# Autodesk Inventor assembly: Trunk
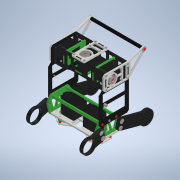
[picture p0: Inventor's stored thumbnail of the model, 180x180]
Saved by Autodesk Inventor 2020.4 (Build 244396000, 396)
## iProperties
Created: 2022-01-05
Part Number: Trunk
Document SubType Name: Assembly
Designer: Masato Kubotera
Mass: 836.462 g
Surface Area: 2738.45 cm^2
Volume: 519.507 cm^3
Density: 1.61011 g/cm^3
Author: Masato Kubotera
## Documents named in this file (24)
- C:\Users\Masato\Desktop\SUSTAINA-OP\UpperBody\Trunk\Trunk.iam
- C:\Users\Masato\Desktop\SUSTAINA-OP\ReadyMade\KONDO\B3M-SC-1170-A.ipt
- C:\Users\Masato\Desktop\SUSTAINA-OP\UpperBody\Trunk\Trunk_chest_frame.ipt
- C:\Users\Masato\Desktop\SUSTAINA-OP\ReadyMade\InsertNut\IRU-304SW.ipt
- C:\Users\Masato\Desktop\SUSTAINA-OP\UpperBody\Trunk\Trunk_neck_frame.ipt
- C:\Users\Masato\Desktop\SUSTAINA-OP\ReadyMade\Screw\M2_6-15.ipt
- C:\Users\Masato\Desktop\SUSTAINA-OP\ReadyMade\Screw\M3-6.ipt
- C:\Users\Masato\Desktop\SUSTAINA-OP\ReadyMade\Screw\M3-8.ipt
- C:\Users\Masato\Desktop\SUSTAINA-OP\UpperBody\Trunk\Trunk_shoulder_frame.ipt
- C:\Users\Masato\Desktop\SUSTAINA-OP\UpperBody\Trunk\Trunk_upper_side_frame.ipt
- C:\Users\Masato\Desktop\SUSTAINA-OP\ReadyMade\Screw\M3-10.ipt
- C:\Users\Masato\Desktop\SUSTAINA-OP\UpperBody\Trunk\Trunk_shoulder_frame_MIR.ipt
- C:\Users\Masato\Desktop\SUSTAINA-OP\ReadyMade\Washer\UUW-0312-10H.ipt
- C:\Users\Masato\Desktop\SUSTAINA-OP\UpperBody\Trunk\Trunk_lower_side_frame.ipt
- C:\Users\Masato\Desktop\SUSTAINA-OP\UpperBody\Trunk\Trunk_waisit_frame.ipt
- C:\Users\Masato\Desktop\SUSTAINA-OP\UpperBody\Trunk\CrossRollerBearing\BearingUnit.iam
- C:\Users\Masato\Desktop\SUSTAINA-OP\ReadyMade\Screw\SPNFL-BRN-M3-6.ipt
- C:\Users\Masato\Desktop\SUSTAINA-OP\ReadyMade\Spacer\ABLSBF7-140-M3-N3.ipt
- C:\Users\Masato\Desktop\SUSTAINA-OP\ReadyMade\Spacer\ABLSBF7-157-M3-N3.ipt
- C:\Users\Masato\Desktop\SUSTAINA-OP\ReadyMade\Spacer\BRU-309S.ipt
- C:\Users\Masato\Desktop\SUSTAINA-OP\UpperBody\Trunk\Trunk_servo_bottom_frame.ipt
- C:\Users\Masato\Desktop\SUSTAINA-OP\ReadyMade\KONDO\B3M-SC-1040-A_with_ClampHorn.iam
- C:\Users\Masato\Desktop\SUSTAINA-OP\UpperBody\Trunk\FrontBumper.ipt
- C:\Users\Masato\Desktop\SUSTAINA-OP\UpperBody\Trunk\RearBumper.ipt
## Components (101 placed, 23 different names)
1. B3M-SC-1170-A:1 — 挿入:87, 挿入:88
2. B3M-SC-1170-A:2 — 挿入:89, 挿入:90
3. Trunk_chest_frame:1 — 挿入:2, 挿入:3, 挿入:4, 挿入:6, 挿入:131
4. Trunk_chest_frame:2 — 挿入:7, 挿入:9, 挿入:10, 挿入:11, 挿入:12, 挿入:8
5. Trunk_neck_frame:1 — 挿入:18, 挿入:20, 挿入:25, 挿入:26, 挿入:27, 挿入:28, 挿入:202, 挿入:203, 挿入:204, 挿入:205
6. Trunk_upper_side_frame:1 — 挿入:29, 挿入:30, 挿入:31, 挿入:32, 挿入:33, 挿入:34, 挿入:35, 挿入:36, 挿入:5, 挿入:119, 挿入:189, 挿入:190, 挿入:193, 挿入:195, 挿入:196
7. Trunk_shoulder_frame:1 — 挿入:33, 挿入:34, 挿入:35, 挿入:36, 挿入:37, 挿入:39, 挿入:38, 挿入:40, 挿入:139, 挿入:200, 挿入:201, 挿入:206, 挿入:207
8. Trunk_upper_side_frame:2 — 挿入:52, 挿入:53, 挿入:54, 挿入:55, 挿入:56, 挿入:57, 挿入:58, 挿入:59, 挿入:120, 挿入:191, 挿入:192, 挿入:194
9. Trunk_shoulder_frame_MIR:1 — 挿入:56, 挿入:57, 挿入:58, 挿入:59, 挿入:65, 挿入:66, 挿入:67, 挿入:68, 挿入:71, 挿入:72, 角度:5, 挿入:141, 挿入:208, 挿入:209
10. UUW-0312-10H:1 — 挿入:75, 挿入:140
11. UUW-0312-10H:2 — 挿入:76, 挿入:142
12. Trunk_lower_side_frame:1 — 挿入:177, 挿入:178, 角度:6, 角度:7, 挿入:179, 挿入:180, 挿入:195, 挿入:196, 挿入:214, 挿入:215, 挿入:216, 挿入:217
13. Trunk_lower_side_frame:2 — 挿入:143, 挿入:144, 挿入:210, 挿入:211, 挿入:212, 挿入:213
14. Trunk_waisit_frame:1 — フラッシュ:2, フラッシュ:3, フラッシュ:4, 挿入:83, 挿入:84, 挿入:85, 挿入:86, 挿入:87, 挿入:88, 挿入:89, 挿入:90, 挿入:91, 挿入:92, 挿入:93, 挿入:94, 挿入:121, 挿入:122, 挿入:123, 挿入:124, 挿入:143, 挿入:144, 挿入:177, 挿入:178
15. BearingUnit:1 [sub-assembly] — 挿入:83, 挿入:84
16. BearingUnit:2 [sub-assembly] — 挿入:85, 挿入:86
17. ABLSBF7-140-M3-N3:1 — 角度:6, 挿入:179
18. ABLSBF7-140-M3-N3:2 — 角度:7, 挿入:180
19. ABLSBF7-157-M3-N3:1 — 角度:5, 挿入:139, 挿入:140, 挿入:141, 挿入:142
20. BRU-309S:1 — 挿入:161, 挿入:214
21. BRU-309S:2 — 挿入:162, 挿入:215
22. BRU-309S:3 — 挿入:163, 挿入:216
23. BRU-309S:4 — 挿入:164, 挿入:217
24. BRU-309S:5 — 挿入:165, 挿入:210
25. BRU-309S:6 — 挿入:166, 挿入:211
26. BRU-309S:7 — 挿入:167, 挿入:212
27. BRU-309S:8 — 挿入:168, 挿入:213
28. UUW-0312-10H:11 — 挿入:161, 挿入:169, 挿入:218
29. UUW-0312-10H:12 — 挿入:162, 挿入:170, 挿入:219
30. UUW-0312-10H:13 — 挿入:163, 挿入:171, 挿入:220
31. UUW-0312-10H:14 — 挿入:164, 挿入:172, 挿入:221
32. UUW-0312-10H:15 — 挿入:165, 挿入:173, 挿入:224
33. UUW-0312-10H:16 — 挿入:166, 挿入:174, 挿入:225
34. UUW-0312-10H:17 — 挿入:167, 挿入:175, 挿入:222
35. UUW-0312-10H:18 — 挿入:168, 挿入:176, 挿入:223
36. Trunk_servo_bottom_frame:1
37. Trunk_servo_bottom_frame:2
38. Trunk_servo_bottom_frame:3
39. M2_6-15:19 — 挿入:202
40. M2_6-15:20 — 挿入:203
41. B3M-SC-1040-A_with_ClampHorn:1 [sub-assembly] — 挿入:204, 挿入:205
42. B3M-SC-1040-A_with_ClampHorn:2 [sub-assembly] — 挿入:206, 挿入:207
43. B3M-SC-1040-A_with_ClampHorn:3 [sub-assembly] — 挿入:208, 挿入:209
44. FrontBumper:1 — 挿入:218, 挿入:219
45. RearBumper:1 — 挿入:220, 挿入:221
46. FrontBumper:2 — 挿入:222, 挿入:223
47. RearBumper:2 — 挿入:224, 挿入:225
48. M2_6-15:17 — 挿入:201
49. M2_6-15:18 — 挿入:200
50. M3-6:9 — 挿入:169
51. M3-6:10 — 挿入:170
52. M3-6:11 — 挿入:171
53. M3-6:12 — 挿入:172
54. M3-6:13 — 挿入:173
55. M3-6:14 — 挿入:174
56. M3-6:15 — 挿入:176
57. M3-6:16 — 挿入:175
58. M3-10:17 — 挿入:189
59. M3-10:18 — 挿入:190
60. M3-10:19 — 挿入:191
61. M3-10:20 — 挿入:192
62. M3-8:7 — 挿入:193
63. M3-8:8 — 挿入:194
64. M3-10:13 — 挿入:121
65. M3-10:14 — 挿入:122
66. M3-10:15 — 挿入:123
67. M3-10:16 — 挿入:124
68. SPNFL-BRN-M3-6:1 — 挿入:119
69. SPNFL-BRN-M3-6:2 — 挿入:120
70. M3-8:2 — 挿入:28
71. M3-8:1 — 挿入:27
72. M3-6:2 — 挿入:26
73. M3-6:1 — 挿入:25
74. M3-8:4 — 挿入:38
75. M3-8:3 — 挿入:37
76. M3-10:4 — 挿入:40
77. M3-10:3 — 挿入:39
78. M2_6-15:12 — 挿入:72
79. M2_6-15:11 — 挿入:71
80. M3-10:6 — 挿入:68
81. M3-10:5 — 挿入:67
82. M3-8:6 — 挿入:66
83. M3-8:5 — 挿入:65
84. M3-6:4 — 挿入:76
85. M3-6:3 — 挿入:75
86. M2_6-15:16 — 挿入:94
87. M2_6-15:15 — 挿入:93
88. M2_6-15:14 — 挿入:92
89. M2_6-15:13 — 挿入:91
90. IRU-304SW:12 — 挿入:12, 挿入:53
91. IRU-304SW:11 — 挿入:11, 挿入:52
92. IRU-304SW:10 — 挿入:10, 挿入:30
93. IRU-304SW:9 — 挿入:9, 挿入:29
94. IRU-304SW:8 — 挿入:8
95. IRU-304SW:7 — 挿入:7, 挿入:18
96. IRU-304SW:6 — 挿入:6, 挿入:32
97. IRU-304SW:5 — 挿入:5, 挿入:31
98. IRU-304SW:4 — 挿入:4, 挿入:55
99. IRU-304SW:3 — 挿入:3, 挿入:54
100. IRU-304SW:2 — 挿入:2, 挿入:20
101. IRU-304SW:1 — 挿入:131
## Relationships (130: Insert 124, Flush 3, Angle 3)
- 挿入:2 [Insert]: Trunk_chest_frame:1 ↔ IRU-304SW:2
- 挿入:3 [Insert]: Trunk_chest_frame:1 ↔ IRU-304SW:3
- 挿入:4 [Insert]: Trunk_chest_frame:1 ↔ IRU-304SW:4
- 挿入:5 [Insert]: Trunk_upper_side_frame:1 ↔ IRU-304SW:5
- 挿入:6 [Insert]: Trunk_chest_frame:1 ↔ IRU-304SW:6
- 挿入:7 [Insert]: Trunk_chest_frame:2 ↔ IRU-304SW:7
- 挿入:8 [Insert]: Trunk_chest_frame:2 ↔ IRU-304SW:8
- 挿入:9 [Insert]: Trunk_chest_frame:2 ↔ IRU-304SW:9
- 挿入:10 [Insert]: Trunk_chest_frame:2 ↔ IRU-304SW:10
- 挿入:11 [Insert]: Trunk_chest_frame:2 ↔ IRU-304SW:11
- 挿入:12 [Insert]: Trunk_chest_frame:2 ↔ IRU-304SW:12
- 挿入:18 [Insert]: Trunk_neck_frame:1 ↔ IRU-304SW:7
- 挿入:20 [Insert]: Trunk_neck_frame:1 ↔ IRU-304SW:2
- 挿入:25 [Insert]: Trunk_neck_frame:1 ↔ M3-6:1
- 挿入:26 [Insert]: Trunk_neck_frame:1 ↔ M3-6:2
- 挿入:27 [Insert]: Trunk_neck_frame:1 ↔ M3-8:1
- 挿入:28 [Insert]: Trunk_neck_frame:1 ↔ M3-8:2
- 挿入:29 [Insert]: Trunk_upper_side_frame:1 ↔ IRU-304SW:9
- 挿入:30 [Insert]: Trunk_upper_side_frame:1 ↔ IRU-304SW:10
- 挿入:31 [Insert]: Trunk_upper_side_frame:1 ↔ IRU-304SW:5
- 挿入:32 [Insert]: Trunk_upper_side_frame:1 ↔ IRU-304SW:6
- 挿入:33 [Insert]: Trunk_upper_side_frame:1 ↔ Trunk_shoulder_frame:1
- 挿入:34 [Insert]: Trunk_upper_side_frame:1 ↔ Trunk_shoulder_frame:1
- 挿入:35 [Insert]: Trunk_upper_side_frame:1 ↔ Trunk_shoulder_frame:1
- 挿入:36 [Insert]: Trunk_upper_side_frame:1 ↔ Trunk_shoulder_frame:1
- 挿入:37 [Insert]: Trunk_shoulder_frame:1 ↔ M3-8:3
- 挿入:39 [Insert]: Trunk_shoulder_frame:1 ↔ M3-10:3
- 挿入:38 [Insert]: Trunk_shoulder_frame:1 ↔ M3-8:4
- 挿入:40 [Insert]: Trunk_shoulder_frame:1 ↔ M3-10:4
- 挿入:52 [Insert]: Trunk_upper_side_frame:2 ↔ IRU-304SW:11
- 挿入:53 [Insert]: Trunk_upper_side_frame:2 ↔ IRU-304SW:12
- 挿入:54 [Insert]: Trunk_upper_side_frame:2 ↔ IRU-304SW:3
- 挿入:55 [Insert]: Trunk_upper_side_frame:2 ↔ IRU-304SW:4
- 挿入:56 [Insert]: Trunk_upper_side_frame:2 ↔ Trunk_shoulder_frame_MIR:1
- 挿入:57 [Insert]: Trunk_upper_side_frame:2 ↔ Trunk_shoulder_frame_MIR:1
- 挿入:58 [Insert]: Trunk_upper_side_frame:2 ↔ Trunk_shoulder_frame_MIR:1
- 挿入:59 [Insert]: Trunk_upper_side_frame:2 ↔ Trunk_shoulder_frame_MIR:1
- 挿入:65 [Insert]: Trunk_shoulder_frame_MIR:1 ↔ M3-8:5
- 挿入:66 [Insert]: Trunk_shoulder_frame_MIR:1 ↔ M3-8:6
- 挿入:67 [Insert]: Trunk_shoulder_frame_MIR:1 ↔ M3-10:5
- 挿入:68 [Insert]: Trunk_shoulder_frame_MIR:1 ↔ M3-10:6
- 挿入:71 [Insert]: Trunk_shoulder_frame_MIR:1 ↔ M2_6-15:11
- 挿入:72 [Insert]: Trunk_shoulder_frame_MIR:1 ↔ M2_6-15:12
- 挿入:75 [Insert]: UUW-0312-10H:1 ↔ M3-6:3
- 挿入:76 [Insert]: UUW-0312-10H:2 ↔ M3-6:4
- フラッシュ:2 [Flush]: Trunk_waisit_frame:1
- フラッシュ:3 [Flush]: Trunk_waisit_frame:1
- フラッシュ:4 [Flush]: Trunk_waisit_frame:1
- 挿入:83 [Insert]: Trunk_waisit_frame:1 ↔ BearingUnit:1
- 挿入:84 [Insert]: Trunk_waisit_frame:1 ↔ BearingUnit:1
- 挿入:85 [Insert]: Trunk_waisit_frame:1 ↔ BearingUnit:2
- 挿入:86 [Insert]: Trunk_waisit_frame:1 ↔ BearingUnit:2
- 挿入:87 [Insert]: B3M-SC-1170-A:1 ↔ Trunk_waisit_frame:1
- 挿入:88 [Insert]: B3M-SC-1170-A:1 ↔ Trunk_waisit_frame:1
- 挿入:89 [Insert]: B3M-SC-1170-A:2 ↔ Trunk_waisit_frame:1
- 挿入:90 [Insert]: B3M-SC-1170-A:2 ↔ Trunk_waisit_frame:1
- 挿入:91 [Insert]: Trunk_waisit_frame:1 ↔ M2_6-15:13
- 挿入:92 [Insert]: Trunk_waisit_frame:1 ↔ M2_6-15:14
- 挿入:93 [Insert]: Trunk_waisit_frame:1 ↔ M2_6-15:15
- 挿入:94 [Insert]: Trunk_waisit_frame:1 ↔ M2_6-15:16
- 挿入:119 [Insert]: Trunk_upper_side_frame:1 ↔ SPNFL-BRN-M3-6:1
- 挿入:120 [Insert]: Trunk_upper_side_frame:2 ↔ SPNFL-BRN-M3-6:2
- 挿入:121 [Insert]: Trunk_waisit_frame:1 ↔ M3-10:13
- 挿入:122 [Insert]: Trunk_waisit_frame:1 ↔ M3-10:14
- 挿入:123 [Insert]: Trunk_waisit_frame:1 ↔ M3-10:15
- 挿入:124 [Insert]: Trunk_waisit_frame:1 ↔ M3-10:16
- 挿入:131 [Insert]: Trunk_chest_frame:1 ↔ IRU-304SW:1
- 角度:5 [Angle] (0 deg): Trunk_shoulder_frame_MIR:1 ↔ ABLSBF7-157-M3-N3:1
- 挿入:139 [Insert]: Trunk_shoulder_frame:1 ↔ ABLSBF7-157-M3-N3:1
- 挿入:140 [Insert]: UUW-0312-10H:1 ↔ ABLSBF7-157-M3-N3:1
- 挿入:141 [Insert]: Trunk_shoulder_frame_MIR:1 ↔ ABLSBF7-157-M3-N3:1
- 挿入:142 [Insert]: UUW-0312-10H:2 ↔ ABLSBF7-157-M3-N3:1
- 挿入:143 [Insert]: Trunk_lower_side_frame:2 ↔ Trunk_waisit_frame:1
- 挿入:144 [Insert]: Trunk_lower_side_frame:2 ↔ Trunk_waisit_frame:1
- 挿入:161 [Insert]: BRU-309S:1 ↔ UUW-0312-10H:11
- 挿入:162 [Insert]: BRU-309S:2 ↔ UUW-0312-10H:12
- 挿入:163 [Insert]: BRU-309S:3 ↔ UUW-0312-10H:13
- 挿入:164 [Insert]: BRU-309S:4 ↔ UUW-0312-10H:14
- 挿入:165 [Insert]: BRU-309S:5 ↔ UUW-0312-10H:15
- 挿入:166 [Insert]: BRU-309S:6 ↔ UUW-0312-10H:16
- 挿入:167 [Insert]: BRU-309S:7 ↔ UUW-0312-10H:17
- 挿入:168 [Insert]: BRU-309S:8 ↔ UUW-0312-10H:18
- 挿入:169 [Insert]: UUW-0312-10H:11 ↔ M3-6:9
- 挿入:170 [Insert]: UUW-0312-10H:12 ↔ M3-6:10
- 挿入:171 [Insert]: UUW-0312-10H:13 ↔ M3-6:11
- 挿入:172 [Insert]: UUW-0312-10H:14 ↔ M3-6:12
- 挿入:173 [Insert]: UUW-0312-10H:15 ↔ M3-6:13
- 挿入:174 [Insert]: UUW-0312-10H:16 ↔ M3-6:14
- 挿入:175 [Insert]: UUW-0312-10H:17 ↔ M3-6:16
- 挿入:176 [Insert]: UUW-0312-10H:18 ↔ M3-6:15
- 挿入:177 [Insert]: Trunk_lower_side_frame:1 ↔ Trunk_waisit_frame:1
- 挿入:178 [Insert]: Trunk_lower_side_frame:1 ↔ Trunk_waisit_frame:1
- 角度:6 [Angle] (0 deg): Trunk_lower_side_frame:1 ↔ ABLSBF7-140-M3-N3:1
- 角度:7 [Angle] (0 deg): Trunk_lower_side_frame:1 ↔ ABLSBF7-140-M3-N3:2
- 挿入:179 [Insert]: Trunk_lower_side_frame:1 ↔ ABLSBF7-140-M3-N3:1
- 挿入:180 [Insert]: Trunk_lower_side_frame:1 ↔ ABLSBF7-140-M3-N3:2
- 挿入:189 [Insert]: Trunk_upper_side_frame:1 ↔ M3-10:17
- 挿入:190 [Insert]: Trunk_upper_side_frame:1 ↔ M3-10:18
- 挿入:191 [Insert]: Trunk_upper_side_frame:2 ↔ M3-10:19
- 挿入:192 [Insert]: Trunk_upper_side_frame:2 ↔ M3-10:20
- 挿入:193 [Insert]: Trunk_upper_side_frame:1 ↔ M3-8:7
- 挿入:194 [Insert]: Trunk_upper_side_frame:2 ↔ M3-8:8
- 挿入:195 [Insert]: Trunk_upper_side_frame:1 ↔ Trunk_lower_side_frame:1
- 挿入:196 [Insert]: Trunk_upper_side_frame:1 ↔ Trunk_lower_side_frame:1
- 挿入:200 [Insert]: Trunk_shoulder_frame:1 ↔ M2_6-15:18
- 挿入:201 [Insert]: Trunk_shoulder_frame:1 ↔ M2_6-15:17
- 挿入:202 [Insert]: Trunk_neck_frame:1 ↔ M2_6-15:19
- 挿入:203 [Insert]: Trunk_neck_frame:1 ↔ M2_6-15:20
- 挿入:204 [Insert]: Trunk_neck_frame:1 ↔ B3M-SC-1040-A_with_ClampHorn:1
- 挿入:205 [Insert]: Trunk_neck_frame:1 ↔ B3M-SC-1040-A_with_ClampHorn:1
- 挿入:206 [Insert]: Trunk_shoulder_frame:1 ↔ B3M-SC-1040-A_with_ClampHorn:2
- 挿入:207 [Insert]: Trunk_shoulder_frame:1 ↔ B3M-SC-1040-A_with_ClampHorn:2
- 挿入:208 [Insert]: Trunk_shoulder_frame_MIR:1 ↔ B3M-SC-1040-A_with_ClampHorn:3
- 挿入:209 [Insert]: Trunk_shoulder_frame_MIR:1 ↔ B3M-SC-1040-A_with_ClampHorn:3
- 挿入:210 [Insert]: Trunk_lower_side_frame:2 ↔ BRU-309S:5
- 挿入:211 [Insert]: Trunk_lower_side_frame:2 ↔ BRU-309S:6
- 挿入:212 [Insert]: Trunk_lower_side_frame:2 ↔ BRU-309S:7
- 挿入:213 [Insert]: Trunk_lower_side_frame:2 ↔ BRU-309S:8
- 挿入:214 [Insert]: Trunk_lower_side_frame:1 ↔ BRU-309S:1
- 挿入:215 [Insert]: Trunk_lower_side_frame:1 ↔ BRU-309S:2
- 挿入:216 [Insert]: Trunk_lower_side_frame:1 ↔ BRU-309S:3
- 挿入:217 [Insert]: Trunk_lower_side_frame:1 ↔ BRU-309S:4
- 挿入:218 [Insert]: UUW-0312-10H:11 ↔ FrontBumper:1
- 挿入:219 [Insert]: UUW-0312-10H:12 ↔ FrontBumper:1
- 挿入:220 [Insert]: UUW-0312-10H:13 ↔ RearBumper:1
- 挿入:221 [Insert]: UUW-0312-10H:14 ↔ RearBumper:1
- 挿入:222 [Insert]: UUW-0312-10H:17 ↔ FrontBumper:2
- 挿入:223 [Insert]: UUW-0312-10H:18 ↔ FrontBumper:2
- 挿入:224 [Insert]: UUW-0312-10H:15 ↔ RearBumper:2
- 挿入:225 [Insert]: UUW-0312-10H:16 ↔ RearBumper:2
